# Autodesk Inventor assembly: BackLowerLink
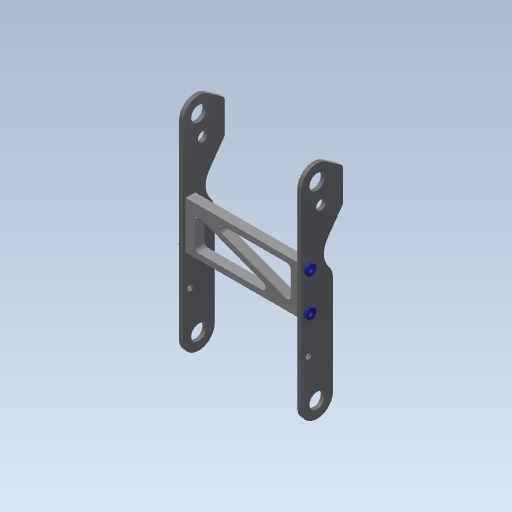
[picture p0: Inventor's stored thumbnail of the model, 512x512]
Saved by Autodesk Inventor 2020.4 (Build 244396000, 396)
## iProperties
Created: 2016-08-23
Part Number: BackLowerLink
Material: 一般
Document SubType Name: Assembly
Designer: hiro
Mass: 27.0677 g
Surface Area: 148.123 cm^2
Volume: 12.1706 cm^3
Density: 2.22402 g/cm^3
Author: hiro
## Documents named in this file (4)
- C:\Users\Masato\Documents\Inventor\CIT Brains_Inventor\OpenPlatform_ver3_0 - ve4_1 branch\LowerBody\Link\BackLowerLink.iam
- C:\Users\Masato\Documents\Inventor\CIT Brains_Inventor\OpenPlatform_ver3_0 - ve4_1 branch\LowerBody\Link\BackLink_diagonal.ipt
- C:\Users\Masato\Documents\Inventor\CIT Brains_Inventor\OpenPlatform_ver3_0 - ve4_1 branch\Ready_Made\Screw\M3-6.ipt
- C:\Users\Masato\Documents\Inventor\CIT Brains_Inventor\OpenPlatform_ver3_0 - ve4_1 branch\LowerBody\Link\BackLink_frame.ipt
## Components (7 placed, 3 different names)
1. BackLink_diagonal:1 — 挿入:31, 挿入:32, 挿入:33, 挿入:34, フラッシュ:1, メイト:1
2. M3-6:1 — 挿入:38
3. M3-6:2 — 挿入:37
4. M3-6:3 — 挿入:41
5. M3-6:4 — 挿入:40
6. BackLink_frame:1 — 挿入:33, 挿入:34, 挿入:37, 挿入:38
7. BackLink_frame:2 — 挿入:31, 挿入:32, 挿入:40, 挿入:41, フラッシュ:2
## Relationships (11: Insert 8, Flush 2, Mate 1)
- 挿入:31 [Insert]: BackLink_diagonal:1 ↔ BackLink_frame:2
- 挿入:32 [Insert]: BackLink_diagonal:1 ↔ BackLink_frame:2
- 挿入:33 [Insert]: BackLink_diagonal:1 ↔ BackLink_frame:1
- 挿入:34 [Insert]: BackLink_diagonal:1 ↔ BackLink_frame:1
- 挿入:37 [Insert]: M3-6:2 ↔ BackLink_frame:1
- 挿入:38 [Insert]: M3-6:1 ↔ BackLink_frame:1
- 挿入:40 [Insert]: M3-6:4 ↔ BackLink_frame:2
- 挿入:41 [Insert]: M3-6:3 ↔ BackLink_frame:2
- フラッシュ:1 [Flush]: BackLink_diagonal:1
- メイト:1 [Mate]: BackLink_diagonal:1
- フラッシュ:2 [Flush]: BackLink_frame:2
